# Autodesk Inventor assembly: Schneekanone
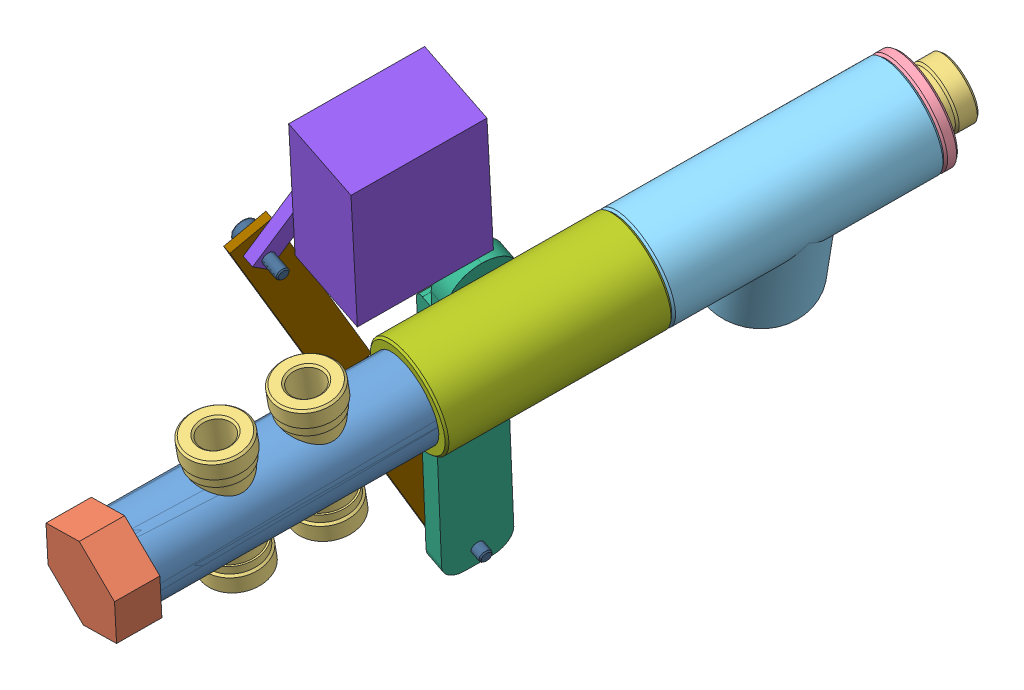
[picture p0: shaded view drawn from the shape stored in the file]
Saved by Autodesk Inventor 2021 (Build 250183000, 183)
## iProperties
Created: 2021-09-01
Part Number: Schneekanone
Document SubType Name: Assembly
Designer: lukas
Author: lukas
## Documents named in this file (36)
- C:\Users\lukas\OneDrive - HTBLA Kaindorf\Diplomarbeit\Mechanik\InventorKonstruktion\Schneekanone.iam
- C:\Users\lukas\OneDrive - HTBLA Kaindorf\Diplomarbeit\Mechanik\InventorKonstruktion\Steher.ipt
- C:\Users\lukas\OneDrive - HTBLA Kaindorf\Diplomarbeit\Mechanik\InventorKonstruktion\Wurfrohr.ipt
- C:\Users\lukas\OneDrive - HTBLA Kaindorf\Diplomarbeit\Mechanik\InventorKonstruktion\BrettSteuereinheit.ipt
- C:\Users\lukas\OneDrive - HTBLA Kaindorf\Diplomarbeit\Mechanik\InventorKonstruktion\Reifen.ipt
- C:\Users\lukas\OneDrive - HTBLA Kaindorf\Diplomarbeit\Mechanik\InventorKonstruktion\SteherStrebe.ipt
- C:\Users\lukas\OneDrive - HTBLA Kaindorf\Diplomarbeit\Mechanik\InventorKonstruktion\Schaltkasten.ipt
- C:\Users\lukas\OneDrive - HTBLA Kaindorf\Diplomarbeit\Mechanik\InventorKonstruktion\WinkelVentilator.ipt
- C:\Users\lukas\OneDrive - HTBLA Kaindorf\Diplomarbeit\Mechanik\InventorKonstruktion\Seitenverkleidung.ipt
- C:\Users\lukas\OneDrive - HTBLA Kaindorf\Diplomarbeit\Mechanik\InventorKonstruktion\Verkleidungsdeckel.ipt
- C:\Users\lukas\OneDrive - HTBLA Kaindorf\Diplomarbeit\Mechanik\InventorKonstruktion\Deckel.ipt
- C:\Users\lukas\OneDrive - HTBLA Kaindorf\Diplomarbeit\Mechanik\InventorKonstruktion\VerteilerLuft1.ipt
- C:\Users\lukas\OneDrive - HTBLA Kaindorf\Diplomarbeit\Mechanik\InventorKonstruktion\VerteilerLuft2.ipt
- C:\Users\lukas\OneDrive - HTBLA Kaindorf\Diplomarbeit\Mechanik\InventorKonstruktion\VentilatorGesamt.iam
- C:\Users\lukas\OneDrive\Documents\Inventor\Content Center Files\R2021\de-DE\IFI 502(60)\IFI 502 - M4x0,7 x 8(8) D.ipt
- C:\Users\lukas\OneDrive\Documents\Inventor\Content Center Files\R2021\de-DE\ISO 7380-1\ISO 7380-1 - M5 x 12.ipt
- C:\Users\lukas\OneDrive\Documents\Inventor\Content Center Files\R2021\de-DE\ANSI B18.2.4.2M\ANSI B18.2.4.2M - M5x0,8 - 8.ipt
- C:\Users\lukas\OneDrive - HTBLA Kaindorf\Diplomarbeit\Mechanik\InventorKonstruktion\Belüftung.ipt
- C:\Users\lukas\OneDrive - HTBLA Kaindorf\Diplomarbeit\Mechanik\InventorKonstruktion\SchlauchAnschluss.ipt
- C:\Users\lukas\OneDrive - HTBLA Kaindorf\Diplomarbeit\Mechanik\InventorKonstruktion\WasserAblauf1.ipt
- C:\Users\lukas\OneDrive - HTBLA Kaindorf\Diplomarbeit\Mechanik\InventorKonstruktion\XPS.ipt
- C:\Users\lukas\OneDrive - HTBLA Kaindorf\Diplomarbeit\Mechanik\InventorKonstruktion\Abdeckungsrohr.ipt
- C:\Users\lukas\OneDrive - HTBLA Kaindorf\Diplomarbeit\Mechanik\InventorKonstruktion\Steuerbares Ventil\1_Default_düse.ipt
- C:\Users\lukas\OneDrive - HTBLA Kaindorf\Diplomarbeit\Mechanik\InventorKonstruktion\Schlauchsteckverbindung.ipt
- C:\Users\lukas\OneDrive - HTBLA Kaindorf\Diplomarbeit\Mechanik\InventorKonstruktion\Nebeldüse.ipt
- C:\Users\lukas\OneDrive - HTBLA Kaindorf\Diplomarbeit\Mechanik\InventorKonstruktion\Wasserverteiler.iam
- C:\Users\lukas\OneDrive - HTBLA Kaindorf\Diplomarbeit\Mechanik\InventorKonstruktion\Durchflusssensor.ipt
- C:\Users\lukas\OneDrive - HTBLA Kaindorf\Diplomarbeit\Mechanik\InventorKonstruktion\Lampe.ipt
- C:\Users\lukas\OneDrive - HTBLA Kaindorf\Diplomarbeit\Mechanik\InventorKonstruktion\Steuerbares Ventil\Ventil.iam
- C:\Users\lukas\OneDrive - HTBLA Kaindorf\Diplomarbeit\Mechanik\InventorKonstruktion\Motor.ipt
- C:\Users\lukas\OneDrive - HTBLA Kaindorf\Diplomarbeit\Mechanik\InventorKonstruktion\Gestänge.ipt
- C:\Users\lukas\OneDrive\Documents\Inventor\Content Center Files\R2021\de-DE\AS 1420\AS 1420 - 1973 - M3 x 8.ipt
- C:\Users\lukas\OneDrive\Documents\Inventor\Content Center Files\R2021\de-DE\ANSI B18.2.4.2M\ANSI B18.2.4.2M - M3x0,5 - 5,5.ipt
- C:\Users\lukas\OneDrive\Documents\Inventor\Content Center Files\R2021\de-DE\AS 1420\AS 1420 - 1973 - M3 x 10.ipt
- C:\Users\lukas\OneDrive - HTBLA Kaindorf\Diplomarbeit\Mechanik\InventorKonstruktion\Steuerbares Ventil\Bedienelement.ipt
- C:\Users\lukas\OneDrive\Documents\Inventor\Content Center Files\R2021\de-DE\IFI 502(00)\IFI 502 - 6.3x1.8 x 13(1) AB I.ipt
## Components (77 placed, 35 different names)
1. Wurfrohr:1 — Drehbar:1, Passend:28, Fluchtend:22, Passend:42, Fluchtend:23, Passend:44, Fluchtend:24, Fluchtend:25, Passend:45, Passend:46, Passend:60, Passend:61, Passend:62, Passend:63, Passend:64, Passend:65, Passend:66, Passend:67, Passend:68, Passend:69, Passend:70, Passend:71, Passend:72, Passend:73, Passend:74, Passend:75, Passend:76, Passend:77, Passend:78, Passend:79, Passend:80, Passend:81, Passend:82, Passend:83, Passend:84, Passend:85, Passend:86, Passend:87, Passend:88, Passend:89, Passend:90, Passend:91, Passend:92, Passend:93, Passend:94, Passend:95
2. BrettSteuereinheit:1 — Passend:8, Fluchtend:10, Passend:21, Passend:27, Passend:102, Passend:103, Fluchtend:28, Passend:104, Passend:105
3. Steher:1 — Passend:6, Fluchtend:8, Fluchtend:9, Drehbar:1, Passend:11, Fluchtend:11, Passend:12, Fluchtend:12, Passend:17, Fluchtend:16, Passend:18, Fluchtend:17, Fluchtend:26, Fluchtend:29, Fluchtend:30
4. Steher:2 — Passend:4, Fluchtend:1, Fluchtend:2, Passend:5, Fluchtend:6, Fluchtend:7, Symmetrie:1, Passend:7, Passend:8, Fluchtend:10, Passend:9, Passend:10, Passend:13, Fluchtend:13, Passend:14, Passend:43, Passend:101, Fluchtend:27, Fluchtend:31
5. SteherStrebe:2 — Passend:4, Fluchtend:1, Fluchtend:2, Fluchtend:9, Passend:21
6. SteherStrebe:4 — Passend:5, Fluchtend:6, Fluchtend:7, Passend:6, Fluchtend:8
7. Reifen:1 — Symmetrie:1, Passend:7
8. Schaltkasten:1 — Passend:9, Passend:10, Passend:19, Passend:20, Passend:22, Passend:23, Passend:37, Passend:38, Passend:39
9. WinkelVentilator:1 — Fluchtend:20, Passend:33, Passend:34, Drehbar:9
10. WinkelVentilator:2 — Fluchtend:21, Passend:35, Passend:36, Drehbar:10
11. WinkelVentilator:3 — Passend:29, Fluchtend:18, Passend:30, Drehbar:7
12. WinkelVentilator:4 — Fluchtend:19, Passend:31, Passend:32, Drehbar:8
13. SteherStrebe:5 — Passend:11, Fluchtend:11, Passend:16, Fluchtend:15, Passend:19, Passend:98, Passend:99, Passend:100
14. SteherStrebe:6 — Passend:12, Fluchtend:12, Passend:20
15. Seitenverkleidung:1 — Passend:13, Fluchtend:13, Passend:14, Passend:15, Fluchtend:14, Passend:109
16. Verkleidungsdeckel:1 — Passend:15, Fluchtend:14, Passend:16, Fluchtend:15
17. Seitenverkleidung:2 — Passend:17, Fluchtend:16, Passend:18
18. Deckel:1 — Passend:22, Passend:23
19. VerteilerLuft1:1 — Starr:1, Starr:2
20. VerteilerLuft2:1 — Starr:2, Passend:27
21. VerteilerLuft2:2 — Starr:1, Fluchtend:17
22. VentilatorGesamt:1 [sub-assembly] — Einfügen:1, Passend:28, Passend:29, Fluchtend:18, Passend:30, Fluchtend:19, Passend:31, Passend:32, Fluchtend:20, Passend:33, Passend:34, Fluchtend:21, Passend:35, Passend:36, Drehbar:3, Drehbar:4, Drehbar:5, Drehbar:6, Fluchtend:22
23. Sechskant Schraube Blechgewinde - Form D - Metrisch M4x0,7 x 8:1 — Einfügen:1
24. ISO 7380-1 M5 x 12:1 — Drehbar:6
25. ISO 7380-1 M5 x 12:2 — Drehbar:3
26. ISO 7380-1 M5 x 12:3 — Drehbar:4
27. ISO 7380-1 M5 x 12:4 — Drehbar:5
28. ANSI B18.2.4.2M M5x0,8:1 — Drehbar:9
29. ANSI B18.2.4.2M M5x0,8:2 — Drehbar:10
30. ANSI B18.2.4.2M M5x0,8:3 — Drehbar:7
31. ANSI B18.2.4.2M M5x0,8:4 — Drehbar:8
32. Belüftung:1 — Passend:37, Passend:38, Passend:39
33. SchlauchAnschluss:1 — Drehbar:13
34. Nebeldüse:11 — Passend:94, Passend:95
35. WasserAblauf1:1 — Passend:42, Fluchtend:23, Passend:43
36. XPS:1 — Passend:44, Fluchtend:24
37. Abdeckungsrohr:1 — Fluchtend:25, Passend:45
38. 1_Default_düse:1 — Passend:46, Drehbar:12, Starr:7, Passend:66
39. 1_Default_düse:5 — Starr:8, Starr:9, Passend:69
40. 1_Default_düse:6 — Starr:3, Starr:4, Passend:60
41. Schlauchsteckverbindung:1 — Starr:3, Passend:62
42. Schlauchsteckverbindung:2 — Starr:4, Passend:61
43. 1_Default_düse:7 — Starr:5, Starr:6, Passend:63
44. Schlauchsteckverbindung:3 — Starr:9, Passend:71
45. Schlauchsteckverbindung:4 — Starr:8, Passend:70
46. Schlauchsteckverbindung:5 — Drehbar:12, Passend:67
47. Schlauchsteckverbindung:6 — Starr:7, Passend:68
48. Schlauchsteckverbindung:7 — Starr:5, Passend:64
49. Schlauchsteckverbindung:8 — Starr:6, Passend:65
50. Nebeldüse:1 — Passend:74, Passend:75
51. Nebeldüse:2 — Passend:72, Passend:73
52. Nebeldüse:4 — Passend:88, Passend:89
53. Nebeldüse:5 — Passend:86, Passend:87
54. Nebeldüse:6 — Passend:84, Passend:85
55. Nebeldüse:7 — Passend:76, Passend:77
56. Nebeldüse:8 — Passend:78, Passend:79
57. Nebeldüse:9 — Passend:82, Passend:83
58. Nebeldüse:10 — Passend:80, Passend:81
59. Nebeldüse:12 — Passend:90, Passend:91
60. Nebeldüse:13 — Passend:92, Passend:93
61. Wasserverteiler:1 [sub-assembly] — Drehbar:14, Passend:102, Fluchtend:26, Drehbar:17, Passend:108
62. Durchflusssensor:1 — Drehbar:13, Drehbar:14
63. Lampe:1 — Passend:98, Passend:99, Passend:100, Passend:101
64. Ventil:1 [sub-assembly] — Passend:103, Fluchtend:27, Fluchtend:28
65. Ventil:2 [sub-assembly] — Passend:104, Fluchtend:29
66. Motor:1 — Passend:105, Fluchtend:30, Passend:106, Drehbar:15
67. Gestänge:1 — Passend:106, Passend:107, Passend:108
68. AS 1420 - Metrisch M3 x 8:2
69. AS 1420 - Metrisch M3 x 10:1 — Drehbar:15, Drehbar:16, Passend:107
70. AS 1420 - Metrisch M3 x 10:2 — Drehbar:17, Drehbar:18
71. ANSI B18.2.4.2M M3x0,5:1 — Drehbar:16
72. ANSI B18.2.4.2M M3x0,5:2 — Drehbar:18
73. Bedienelement:1 — Passend:109, Fluchtend:31, Drehbar:19, Drehbar:20, Drehbar:21, Drehbar:22
74. Linsensenkkopf-Blechschraube mit Kreuzschlitz - Form AB - Typ I - Metrisch (IFI) 6.3x1.8 x 13:1 — Drehbar:19
75. Linsensenkkopf-Blechschraube mit Kreuzschlitz - Form AB - Typ I - Metrisch (IFI) 6.3x1.8 x 13:2 — Drehbar:20
76. Linsensenkkopf-Blechschraube mit Kreuzschlitz - Form AB - Typ I - Metrisch (IFI) 6.3x1.8 x 13:3 — Drehbar:22
77. Linsensenkkopf-Blechschraube mit Kreuzschlitz - Form AB - Typ I - Metrisch (IFI) 6.3x1.8 x 13:4 — Drehbar:21
## Relationships (145: Mate 86, Flush 28, RevoluteJoint 20, WeldJoint 9, Symmetry 1, Insert 1)
- Passend:4 [Mate]: Steher:2 ↔ SteherStrebe:2
- Fluchtend:1 [Flush]: Steher:2 ↔ SteherStrebe:2
- Fluchtend:2 [Flush] (233.058 mm): Steher:2 ↔ SteherStrebe:2
- Passend:5 [Mate]: Steher:2 ↔ SteherStrebe:4
- Fluchtend:6 [Flush]: Steher:2 ↔ SteherStrebe:4
- Fluchtend:7 [Flush] (308.058 mm): Steher:2 ↔ SteherStrebe:4
- Passend:6 [Mate]: Steher:1 ↔ SteherStrebe:4
- Fluchtend:8 [Flush]: Steher:1 ↔ SteherStrebe:4
- Fluchtend:9 [Flush]: Steher:1 ↔ SteherStrebe:2
- Symmetrie:1: Steher:2 ↔ Reifen:1
- Passend:7 [Mate] (10 mm): Steher:2 ↔ Reifen:1
- Passend:8 [Mate]: BrettSteuereinheit:1 ↔ Steher:2
- Fluchtend:10 [Flush]: BrettSteuereinheit:1 ↔ Steher:2
- Drehbar:1 [RevoluteJoint] (-10 mm): Wurfrohr:1 ↔ Steher:1
- Passend:9 [Mate] (2.5 mm): Steher:2 ↔ Schaltkasten:1
- Passend:10 [Mate]: Steher:2 ↔ Schaltkasten:1
- Passend:11 [Mate]: Steher:1 ↔ SteherStrebe:5
- Fluchtend:11 [Flush]: Steher:1 ↔ SteherStrebe:5
- Passend:12 [Mate]: Steher:1 ↔ SteherStrebe:6
- Fluchtend:12 [Flush]: Steher:1 ↔ SteherStrebe:6
- Passend:13 [Mate]: Steher:2 ↔ Seitenverkleidung:1
- Fluchtend:13 [Flush]: Steher:2 ↔ Seitenverkleidung:1
- Passend:14 [Mate]: Steher:2 ↔ Seitenverkleidung:1
- Passend:15 [Mate]: Seitenverkleidung:1 ↔ Verkleidungsdeckel:1
- Fluchtend:14 [Flush]: Seitenverkleidung:1 ↔ Verkleidungsdeckel:1
- Passend:16 [Mate]: SteherStrebe:5 ↔ Verkleidungsdeckel:1
- Fluchtend:15 [Flush]: SteherStrebe:5 ↔ Verkleidungsdeckel:1
- Passend:17 [Mate]: Steher:1 ↔ Seitenverkleidung:2
- Fluchtend:16 [Flush]: Steher:1 ↔ Seitenverkleidung:2
- Passend:18 [Mate]: Steher:1 ↔ Seitenverkleidung:2
- Passend:19 [Mate] (2 mm): Schaltkasten:1 ↔ SteherStrebe:5
- Passend:20 [Mate] (2 mm): Schaltkasten:1 ↔ SteherStrebe:6
- Passend:21 [Mate] (477 mm): BrettSteuereinheit:1 ↔ SteherStrebe:2
- Passend:22 [Mate]: Schaltkasten:1 ↔ Deckel:1
- Passend:23 [Mate]: Schaltkasten:1 ↔ Deckel:1
- Starr:1 [WeldJoint]: VerteilerLuft1:1 ↔ VerteilerLuft2:2
- Starr:2 [WeldJoint]: VerteilerLuft1:1 ↔ VerteilerLuft2:1
- Passend:27 [Mate]: BrettSteuereinheit:1 ↔ VerteilerLuft2:1
- Fluchtend:17 [Flush] (120 mm): Steher:1 ↔ VerteilerLuft2:2
- Einfügen:1 [Insert]: VentilatorGesamt:1 ↔ Sechskant Schraube Blechgewinde - Form D - Metrisch M4x0,7 x 8:1
- Passend:28 [Mate]: Wurfrohr:1 ↔ VentilatorGesamt:1
- Passend:29 [Mate]: WinkelVentilator:3 ↔ VentilatorGesamt:1
- Fluchtend:18 [Flush]: WinkelVentilator:3 ↔ VentilatorGesamt:1
- Passend:30 [Mate] (7 mm): WinkelVentilator:3 ↔ VentilatorGesamt:1
- Fluchtend:19 [Flush]: WinkelVentilator:4 ↔ VentilatorGesamt:1
- Passend:31 [Mate]: WinkelVentilator:4 ↔ VentilatorGesamt:1
- Passend:32 [Mate] (7 mm): WinkelVentilator:4 ↔ VentilatorGesamt:1
- Fluchtend:20 [Flush]: WinkelVentilator:1 ↔ VentilatorGesamt:1
- Passend:33 [Mate]: WinkelVentilator:1 ↔ VentilatorGesamt:1
- Passend:34 [Mate] (7 mm): WinkelVentilator:1 ↔ VentilatorGesamt:1
- Fluchtend:21 [Flush]: WinkelVentilator:2 ↔ VentilatorGesamt:1
- Passend:35 [Mate]: WinkelVentilator:2 ↔ VentilatorGesamt:1
- Passend:36 [Mate] (7 mm): WinkelVentilator:2 ↔ VentilatorGesamt:1
- Drehbar:3 [RevoluteJoint]: VentilatorGesamt:1 ↔ ISO 7380-1 M5 x 12:2
- Drehbar:4 [RevoluteJoint]: VentilatorGesamt:1 ↔ ISO 7380-1 M5 x 12:3
- Drehbar:5 [RevoluteJoint]: VentilatorGesamt:1 ↔ ISO 7380-1 M5 x 12:4
- Drehbar:6 [RevoluteJoint]: VentilatorGesamt:1 ↔ ISO 7380-1 M5 x 12:1
- Drehbar:7 [RevoluteJoint]: WinkelVentilator:3 ↔ ANSI B18.2.4.2M M5x0,8:3
- Drehbar:8 [RevoluteJoint]: WinkelVentilator:4 ↔ ANSI B18.2.4.2M M5x0,8:4
- Drehbar:9 [RevoluteJoint]: WinkelVentilator:1 ↔ ANSI B18.2.4.2M M5x0,8:1
- Drehbar:10 [RevoluteJoint]: WinkelVentilator:2 ↔ ANSI B18.2.4.2M M5x0,8:2
- Fluchtend:22 [Flush] (-20 mm): Wurfrohr:1 ↔ VentilatorGesamt:1
- Passend:37 [Mate]: Schaltkasten:1 ↔ Belüftung:1
- Passend:38 [Mate]: Schaltkasten:1 ↔ Belüftung:1
- Passend:39 [Mate]: Schaltkasten:1 ↔ Belüftung:1
- Passend:42 [Mate]: Wurfrohr:1 ↔ WasserAblauf1:1
- Fluchtend:23 [Flush] (200 mm): Wurfrohr:1 ↔ WasserAblauf1:1
- Passend:43 [Mate] (162 mm): Steher:2 ↔ WasserAblauf1:1
- Passend:44 [Mate]: Wurfrohr:1 ↔ XPS:1
- Fluchtend:24 [Flush] (150 mm): Wurfrohr:1 ↔ XPS:1
- Fluchtend:25 [Flush]: Wurfrohr:1 ↔ Abdeckungsrohr:1
- Passend:45 [Mate]: Wurfrohr:1 ↔ Abdeckungsrohr:1
- Passend:46 [Mate]: Wurfrohr:1 ↔ 1_Default_düse:1
- Starr:3 [WeldJoint] (-8 mm): 1_Default_düse:6 ↔ Schlauchsteckverbindung:1
- Starr:4 [WeldJoint] (-8 mm): 1_Default_düse:6 ↔ Schlauchsteckverbindung:2
- Passend:60 [Mate]: Wurfrohr:1 ↔ 1_Default_düse:6
- Passend:61 [Mate]: Wurfrohr:1 ↔ Schlauchsteckverbindung:2
- Passend:62 [Mate]: Wurfrohr:1 ↔ Schlauchsteckverbindung:1
- Starr:5 [WeldJoint] (8 mm): 1_Default_düse:7 ↔ Schlauchsteckverbindung:7
- Starr:6 [WeldJoint] (-8 mm): 1_Default_düse:7 ↔ Schlauchsteckverbindung:8
- Passend:63 [Mate]: Wurfrohr:1 ↔ 1_Default_düse:7
- Passend:64 [Mate]: Wurfrohr:1 ↔ Schlauchsteckverbindung:7
- Passend:65 [Mate]: Wurfrohr:1 ↔ Schlauchsteckverbindung:8
- Drehbar:12 [RevoluteJoint] (8 mm): 1_Default_düse:1 ↔ Schlauchsteckverbindung:5
- Starr:7 [WeldJoint] (-8 mm): 1_Default_düse:1 ↔ Schlauchsteckverbindung:6
- Passend:66 [Mate]: Wurfrohr:1 ↔ 1_Default_düse:1
- Passend:67 [Mate]: Wurfrohr:1 ↔ Schlauchsteckverbindung:5
- Passend:68 [Mate]: Wurfrohr:1 ↔ Schlauchsteckverbindung:6
- Starr:8 [WeldJoint] (-8 mm): 1_Default_düse:5 ↔ Schlauchsteckverbindung:4
- Starr:9 [WeldJoint] (-8 mm): 1_Default_düse:5 ↔ Schlauchsteckverbindung:3
- Passend:69 [Mate]: Wurfrohr:1 ↔ 1_Default_düse:5
- Passend:70 [Mate]: Wurfrohr:1 ↔ Schlauchsteckverbindung:4
- Passend:71 [Mate]: Wurfrohr:1 ↔ Schlauchsteckverbindung:3
- Passend:72 [Mate]: Wurfrohr:1 ↔ Nebeldüse:2
- Passend:73 [Mate]: Wurfrohr:1 ↔ Nebeldüse:2
- Passend:74 [Mate]: Wurfrohr:1 ↔ Nebeldüse:1
- Passend:75 [Mate]: Wurfrohr:1 ↔ Nebeldüse:1
- Passend:76 [Mate]: Wurfrohr:1 ↔ Nebeldüse:7
- Passend:77 [Mate]: Wurfrohr:1 ↔ Nebeldüse:7
- Passend:78 [Mate]: Wurfrohr:1 ↔ Nebeldüse:8
- Passend:79 [Mate]: Wurfrohr:1 ↔ Nebeldüse:8
- Passend:80 [Mate]: Wurfrohr:1 ↔ Nebeldüse:10
- Passend:81 [Mate]: Wurfrohr:1 ↔ Nebeldüse:10
- Passend:82 [Mate]: Wurfrohr:1 ↔ Nebeldüse:9
- Passend:83 [Mate]: Wurfrohr:1 ↔ Nebeldüse:9
- Passend:84 [Mate]: Wurfrohr:1 ↔ Nebeldüse:6
- Passend:85 [Mate]: Wurfrohr:1 ↔ Nebeldüse:6
- Passend:86 [Mate]: Wurfrohr:1 ↔ Nebeldüse:5
- Passend:87 [Mate]: Wurfrohr:1 ↔ Nebeldüse:5
- Passend:88 [Mate]: Wurfrohr:1 ↔ Nebeldüse:4
- Passend:89 [Mate]: Wurfrohr:1 ↔ Nebeldüse:4
- Passend:90 [Mate]: Wurfrohr:1 ↔ Nebeldüse:12
- Passend:91 [Mate]: Wurfrohr:1 ↔ Nebeldüse:12
- Passend:92 [Mate]: Wurfrohr:1 ↔ Nebeldüse:13
- Passend:93 [Mate]: Wurfrohr:1 ↔ Nebeldüse:13
- Passend:94 [Mate]: Wurfrohr:1 ↔ Nebeldüse:11
- Passend:95 [Mate]: Wurfrohr:1 ↔ Nebeldüse:11
- Drehbar:13 [RevoluteJoint] (-10 mm): SchlauchAnschluss:1 ↔ Durchflusssensor:1
- Drehbar:14 [RevoluteJoint] (-10 mm): Wasserverteiler:1 ↔ Durchflusssensor:1
- Passend:98 [Mate]: SteherStrebe:5 ↔ Lampe:1
- Passend:99 [Mate]: SteherStrebe:5 ↔ Lampe:1
- Passend:100 [Mate] (15 mm): SteherStrebe:5 ↔ Lampe:1
- Passend:101 [Mate] (187 mm): Steher:2 ↔ Lampe:1
- Passend:102 [Mate]: BrettSteuereinheit:1 ↔ Wasserverteiler:1
- Fluchtend:26 [Flush] (125 mm): Steher:1 ↔ Wasserverteiler:1
- Passend:103 [Mate] (-5 mm): BrettSteuereinheit:1 ↔ Ventil:1
- Fluchtend:27 [Flush] (-50 mm): Steher:2 ↔ Ventil:1
- Fluchtend:28 [Flush] (230 mm): BrettSteuereinheit:1 ↔ Ventil:1
- Passend:104 [Mate] (-5 mm): BrettSteuereinheit:1 ↔ Ventil:2
- Fluchtend:29 [Flush] (50 mm): Steher:1 ↔ Ventil:2
- Passend:105 [Mate]: BrettSteuereinheit:1 ↔ Motor:1
- Fluchtend:30 [Flush] (180 mm): Steher:1 ↔ Motor:1
- Passend:106 [Mate]: Motor:1 ↔ Gestänge:1
- Drehbar:15 [RevoluteJoint] (7.5 mm): Motor:1 ↔ AS 1420 - Metrisch M3 x 10:1
- Drehbar:16 [RevoluteJoint] (-4.5 mm): AS 1420 - Metrisch M3 x 10:1 ↔ ANSI B18.2.4.2M M3x0,5:1
- Passend:107 [Mate]: Gestänge:1 ↔ AS 1420 - Metrisch M3 x 10:1
- Drehbar:17 [RevoluteJoint] (7.5 mm): Wasserverteiler:1 ↔ AS 1420 - Metrisch M3 x 10:2
- Drehbar:18 [RevoluteJoint]: AS 1420 - Metrisch M3 x 10:2 ↔ ANSI B18.2.4.2M M3x0,5:2
- Passend:108 [Mate]: Wasserverteiler:1 ↔ Gestänge:1
- Passend:109 [Mate]: Seitenverkleidung:1 ↔ Bedienelement:1
- Fluchtend:31 [Flush] (65 mm): Steher:2 ↔ Bedienelement:1
- Drehbar:19 [RevoluteJoint] (4 mm): Bedienelement:1 ↔ Linsensenkkopf-Blechschraube mit Kreuzschlitz - Form AB - Typ I - Metrisch (IFI) 6.3x1.8 x 13:1
- Drehbar:20 [RevoluteJoint] (4 mm): Bedienelement:1 ↔ Linsensenkkopf-Blechschraube mit Kreuzschlitz - Form AB - Typ I - Metrisch (IFI) 6.3x1.8 x 13:2
- Drehbar:21 [RevoluteJoint] (4 mm): Bedienelement:1 ↔ Linsensenkkopf-Blechschraube mit Kreuzschlitz - Form AB - Typ I - Metrisch (IFI) 6.3x1.8 x 13:4
- Drehbar:22 [RevoluteJoint] (4 mm): Bedienelement:1 ↔ Linsensenkkopf-Blechschraube mit Kreuzschlitz - Form AB - Typ I - Metrisch (IFI) 6.3x1.8 x 13:3
